# Autodesk Inventor assembly: Corrected Side Plate Assembly V2
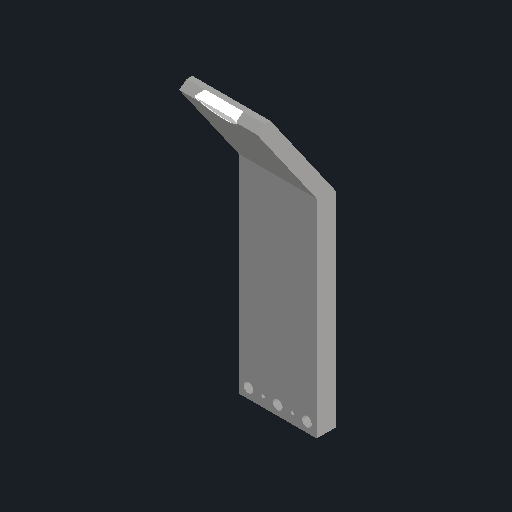
[picture p0: Inventor's stored thumbnail of the model, 512x512]
Saved by Autodesk Inventor 2026 (Build 300175000, 175)
## iProperties
Created: 2026-03-17
Part Number: Corrected Side Plate Assembly V2
Document SubType Name: Assembly
Designer: FiolkaLab
Author: FiolkaLab
## Documents named in this file (3)
- E:\Muaaz\Baseplate\Illumination\Corrected Side Plate Assembly V2.iam
- E:\Muaaz\Baseplate\Illumination\PFD10-03-P01-Step\PFD10-03-P01-Step\PFD10-03-P01-Step.ipt
- E:\Muaaz\Baseplate\Illumination\Side plate for Inclined Mirror D shaped V2.ipt
## Components (2 placed, 2 different names)
1. PFD10-03-P01-Step:1 — Mate:1, Mate:2
2. Side plate for Inclined Mirror D shaped V2:1 — Mate:1, Mate:2
## Relationships (2: Mate 2)
- Mate:1: PFD10-03-P01-Step:1 ↔ Side plate for Inclined Mirror D shaped V2:1
- Mate:2: PFD10-03-P01-Step:1 ↔ Side plate for Inclined Mirror D shaped V2:1
